# Autodesk Inventor assembly: motor_MIR
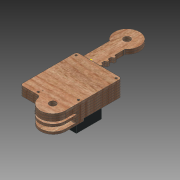
[picture p0: Inventor's stored thumbnail of the model, 180x180]
Saved by Autodesk Inventor 2015 (Build 190159000, 159)
## iProperties
Created: 2016-02-03
Part Number: motor_MIR
Document SubType Name: Assembly
Designer: david
Author: david
## Documents named in this file (11)
- Z:\gip\Inventor\generatie 7\motor\motor_MIR.iam
- Z:\gip\Inventor\generatie 7\motor\p1.ipt
- Z:\gip\Inventor\generatie 7\motor\p2_MIR.ipt
- Z:\gip\Inventor\generatie 7\motor\p3_MIR.ipt
- Z:\gip\Inventor\generatie 7\motor\p4_MIR.ipt
- Z:\gip\Inventor\generatie 7\motor\p5_MIR.ipt
- Z:\gip\Inventor\generatie 7\motor\servo\block_MIR1.ipt
- Z:\gip\Inventor\generatie 7\motor\servo\tang_MIR.ipt
- Z:\gip\Inventor\generatie 7\old\Motor\tanden_MIR.ipt
- Z:\gip\Inventor\generatie 7\motor\tandwiel\tandwiel_MIR.iam
- Z:\gip\Inventor\generatie 7\motor\p6_MIR.ipt
## Components (13 placed, 10 different names)
1. p1:1 — Flush:2, Flush:1, Mate:1, Flush:4
2. p2_MIR:1 — Flush:2, Flush:1, Mate:1, Flush:3, Mate:2, Flush:5, Mate:21
3. p2_MIR:2 — Flush:4, Flush:3, Mate:2, Flush:6, Mate:3, Mate:15, Mate:14
4. p3_MIR:1 — Flush:6, Flush:5, Mate:3, Mate:5, Flush:8, Flush:7, Mate:13
5. p4_MIR:1 — Mate:5, Flush:8, Flush:7, Mate:6, Flush:10, Flush:9
6. p5_MIR:1 — Mate:6, Flush:10, Flush:9, Mate:7, Flush:12, Flush:11, Mate:17
7. p5_MIR:2 — Mate:7, Flush:12, Flush:11, Mate:12, Mate:9, Mate:8, Flush:14
8. block_MIR1:1 — Mate:12, Mate:9, Mate:8, Mate:11, Mate:10
9. tang_MIR:1 — Mate:11, Mate:10, Mate:18, Mate:16
10. tanden_MIR:1 — Mate:15, Mate:14, Mate:13, Rotation/Translation:1, Mate:20, Flush:13, Mate:19, Mate:21
11. tandwiel_MIR:1 [sub-assembly] — Mate:18, Mate:17, Mate:16, Rotation/Translation:1
12. tanden_MIR:2 — Mate:20, Flush:13, Mate:19
13. p6_MIR:1 — Flush:14
## Relationships (35: Mate 21, Flush 13, RelateRotateTranslate 1)
- Flush:2: p1:1 ↔ p2_MIR:1
- Flush:1: p1:1 ↔ p2_MIR:1
- Mate:1: p1:1 ↔ p2_MIR:1
- Flush:4: p1:1 ↔ p2_MIR:2
- Flush:3: p2_MIR:1 ↔ p2_MIR:2
- Mate:2: p2_MIR:1 ↔ p2_MIR:2
- Flush:6: p2_MIR:2 ↔ p3_MIR:1
- Flush:5: p2_MIR:1 ↔ p3_MIR:1
- Mate:3: p2_MIR:2 ↔ p3_MIR:1
- Mate:5: p3_MIR:1 ↔ p4_MIR:1
- Flush:8: p3_MIR:1 ↔ p4_MIR:1
- Flush:7: p3_MIR:1 ↔ p4_MIR:1
- Mate:6: p4_MIR:1 ↔ p5_MIR:1
- Flush:10: p4_MIR:1 ↔ p5_MIR:1
- Flush:9: p4_MIR:1 ↔ p5_MIR:1
- Mate:7: p5_MIR:1 ↔ p5_MIR:2
- Flush:12: p5_MIR:1 ↔ p5_MIR:2
- Flush:11: p5_MIR:1 ↔ p5_MIR:2
- Mate:12: p5_MIR:2 ↔ block_MIR1:1
- Mate:9: p5_MIR:2 ↔ block_MIR1:1
- Mate:8: p5_MIR:2 ↔ block_MIR1:1
- Mate:11: block_MIR1:1 ↔ tang_MIR:1
- Mate:10: block_MIR1:1 ↔ tang_MIR:1
- Mate:15: p2_MIR:2 ↔ tanden_MIR:1
- Mate:14: p2_MIR:2 ↔ tanden_MIR:1
- Mate:13: p3_MIR:1 ↔ tanden_MIR:1
- Mate:18: tang_MIR:1 ↔ tandwiel_MIR:1
- Mate:17: p5_MIR:1 ↔ tandwiel_MIR:1
- Mate:16 (0.15 mm): tang_MIR:1 ↔ tandwiel_MIR:1
- Rotation/Translation:1 [RelateRotateTranslate] (100 mm): tanden_MIR:1 ↔ tandwiel_MIR:1
- Mate:20: tanden_MIR:1 ↔ tanden_MIR:2
- Flush:13: tanden_MIR:1 ↔ tanden_MIR:2
- Mate:19: tanden_MIR:1 ↔ tanden_MIR:2
- Flush:14 [Mate]: p5_MIR:2 ↔ p6_MIR:1
- Mate:21: p2_MIR:1 ↔ tanden_MIR:1
